# Autodesk Inventor assembly: CrossBot
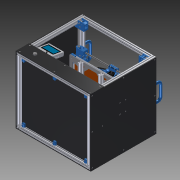
[picture p0: Inventor's stored thumbnail of the model, 180x180]
Saved by Autodesk Inventor 2015 SP1 (Build 190203100, 203)
## iProperties
Created: 2014-08-14
Part Number: CrossBot
Document SubType Name: Assembly
Designer: t_clevj
Mass: 16815.8 g
Surface Area: 53062.5 cm^2
Volume: 10946.1 cm^3
Density: 1.53623 g/cm^3
Author: t_clevj
## Documents named in this file (25)
- C:\Users\Jack\ownCloud\Projects\CrossBot\InventorModel\CrossBot.iam
- C:\Users\Jack\ownCloud\Projects\CrossBot\InventorModel\Frame\Frame.iam
- C:\Users\Jack\ownCloud\Projects\CrossBot\InventorModel\Hardware\Shaft\Shaft8\YShaft.ipt
- C:\Users\Jack\ownCloud\Projects\CrossBot\InventorModel\YAxis\YAxisMotorLeft.iam
- C:\Users\Jack\ownCloud\Projects\CrossBot\InventorModel\YAxis\YAxisIdlerLeft.iam
- C:\Users\Jack\ownCloud\Projects\CrossBot\InventorModel\YAxis\YAxisMotorRight.iam
- C:\Users\Jack\ownCloud\Projects\CrossBot\InventorModel\XAxis\XEndLeft.iam
- C:\Users\Jack\ownCloud\Projects\CrossBot\InventorModel\YAxis\YAxisIdlerRight.iam
- C:\Users\Jack\ownCloud\Projects\CrossBot\InventorModel\XAxis\XEndRight.iam
- C:\Users\Jack\ownCloud\Projects\CrossBot\InventorModel\Hardware\Shaft\Shaft8\XShaft.ipt
- C:\Users\Jack\ownCloud\Projects\CrossBot\InventorModel\Hardware\Shaft\Shaft10\ZAxisShaft.ipt
- C:\Users\Jack\ownCloud\Projects\CrossBot\InventorModel\Enclosure\SpoolFilament.ipt
- C:\Users\Jack\ownCloud\Projects\CrossBot\InventorModel\XAxis\XCarriage.iam
- C:\Users\Jack\ownCloud\Projects\CrossBot\InventorModel\Electronics\PSUUltibots.ipt
- C:\Users\Jack\ownCloud\Projects\CrossBot\InventorModel\Extruder\SanladererBowdenExtruder\SanladererBowdenExtruder.iam
- C:\Users\Jack\ownCloud\Projects\CrossBot\InventorModel\Extruder\SanladererBowdenExtruder\SanladererBowdenExtruderMirrored.iam
- C:\Users\Jack\ownCloud\Projects\CrossBot\InventorModel\ZAxis\ZAxisBed.iam
- C:\Users\Jack\ownCloud\Projects\CrossBot\InventorModel\ZAxis\ZAxisRodClamp.iam
- C:\Users\Jack\ownCloud\Projects\CrossBot\InventorModel\ZAxis\ZDrive.iam
- C:\Users\Jack\ownCloud\Projects\CrossBot\InventorModel\Electronics\KeySwitch\KeySwitch.iam
- C:\Users\Jack\ownCloud\Projects\CrossBot\InventorModel\ZAxis\ZEndstop.iam
- C:\Users\Jack\ownCloud\Projects\CrossBot\InventorModel\Electronics\Ports\PowerSocket.ipt
- C:\Users\Jack\ownCloud\Projects\CrossBot\InventorModel\Hardware\Nuts\ExtrusionNuts\ExtrusionNutHNKK5_4.ipt
- C:\Users\Jack\ownCloud\Projects\CrossBot\InventorModel\Electronics\Boards\RumbaBoard.ipt
- C:\Users\Jack\ownCloud\Projects\CrossBot\InventorModel\Enclosure\LCDCase\LCD+Case.iam
## Components (60 placed, 24 different names)
1. Frame:1 [sub-assembly] — Mate:6, Mate:23, Mate:24, Mate:25, Mate:27, Mate:28, Mate:29, Mate:30, Mate:31, Mate:32, Mate:69, Mate:70, Angle:13, Mate:260, Flush:89, Mate:261, Flush:90, Flush:92, Flush:93, Flush:94, Flush:95, Mate:352, Mate:353, Mate:354, Mate:355, Flush:98, Mate:381, Mate:382, Mate:383, Mate:400, Mate:401, Mate:402, Angle:46, Mate:417, Mate:418, Mate:419, Mate:426, Mate:427, Mate:428, Angle:47, Mate:465, Angle:50, Angle:51, Angle:52, Angle:53, Angle:54, Angle:55, Mate:466, Mate:467, Mate:468, Mate:469, Mate:470, Angle:56, Angle:58, Angle:59, Angle:60, Angle:61, Angle:62, Angle:63, Angle:64, Angle:65, Angle:66, Mate:471, Mate:472, Mate:473, Mate:474, Mate:475, Mate:476, Mate:477, Mate:478, Mate:479, Mate:480, Angle:67, Angle:68, Angle:69, Angle:70, Mate:481, Mate:482, Mate:483, Mate:484, Angle:71, Angle:72, Angle:73, Angle:74, Mate:485, Mate:486, Mate:487, Mate:488, Angle:75, Angle:76, Angle:77, Angle:78, Mate:489, Mate:490, Mate:491, Mate:492, Mate:497, Mate:498, Mate:499, Angle:79
2. RumbaBoard:1 — Mate:498
3. LCD+Case:1 [sub-assembly] — Mate:499, Angle:79
4. ZEndstop:1 [sub-assembly] — Mate:415, Angle:46, Mate:416
5. ZDrive:1 [sub-assembly] — Mate:381, Mate:382, Mate:383, Mate:384, Mate:431, Mate:459, Mate:460, Mate:461, Mate:462
6. ZAxisRodClamp:4 [sub-assembly] — Mate:350, Flush:95, Mate:355, Mate:384, Mate:455, Mate:456
7. ZAxisRodClamp:3 [sub-assembly] — Mate:349, Flush:94, Mate:352, Flush:97, Mate:416, Mate:463, Mate:464
8. ZAxisRodClamp:2 [sub-assembly] — Mate:348, Flush:92, Mate:354, Mate:457, Mate:458
9. ZAxisRodClamp:1 [sub-assembly] — Mate:347, Flush:93, Mate:353, Flush:96, Mate:449, Mate:450
10. ZAxisBed:1 [sub-assembly] — Mate:431, Angle:47
11. ZAxisShaft:1 — Mate:349, Mate:350, Mate:351, Flush:97, Mate:415
12. ZAxisShaft:2 — Mate:347, Mate:348, Mate:351, Flush:96
13. YShaft:2 — Mate:26, Mate:130, Mate:514
14. YShaft:3 — Mate:37, Mate:190
15. YAxisMotorLeft:1 [sub-assembly] — Mate:23, Mate:24, Mate:25, Mate:26, Mate:439, Mate:440, Mate:441, Mate:442
16. YAxisMotorRight:1 [sub-assembly] — Mate:30, Mate:31, Mate:32, Mate:37, Mate:435, Mate:436, Mate:437, Mate:438
17. YAxisIdlerLeft:1 [sub-assembly] — Mate:27, Mate:28, Mate:29, Mate:130, Mate:443, Mate:444, Mate:445
18. YAxisIdlerRight:1 [sub-assembly] — Mate:426, Mate:427, Mate:428, Mate:446, Mate:447, Mate:448
19. XShaft:1 — Mate:189, Flush:54, Mate:513, Mate:515
20. XShaft:2 — Mate:188, Flush:55, Mate:191, Mate:516
21. XCarriage:1 [sub-assembly] — Mate:515, Mate:516
22. XEndLeft:1 [sub-assembly] — Mate:188, Mate:189, Flush:54, Flush:55, Mate:514
23. XEndRight:1 [sub-assembly] — Mate:190, Mate:191, Angle:13, Mate:513
24. KeySwitch:1 [sub-assembly] — Mate:400, Mate:401, Mate:402
25. PowerSocket:1 — Mate:417, Mate:418, Mate:419
26. PSUUltibots:1 — Mate:497
27. SpoolFilament:3 — Mate:504
28. SpoolFilament:4 — Mate:504
29. SanladererBowdenExtruderMirrored:1 [sub-assembly] — Mate:261, Flush:90, Flush:91, Mate:493, Mate:494
30. SanladererBowdenExtruder:1 [sub-assembly] — Mate:260, Flush:89, Flush:91, Flush:98, Mate:495, Mate:496
31. ExtrusionNutHNKK5_4:22 — Mate:455, Angle:51, Mate:469
32. ExtrusionNutHNKK5_4:30 — Mate:464, Angle:74, Mate:485
33. ExtrusionNutHNKK5_4:29 — Mate:463, Angle:71, Mate:486
34. ExtrusionNutHNKK5_4:16 — Mate:450, Angle:73, Mate:487
35. ExtrusionNutHNKK5_4:15 — Mate:449, Angle:72, Mate:488
36. ExtrusionNutHNKK5_4:23 — Mate:457, Angle:53, Mate:466
37. ExtrusionNutHNKK5_4:24 — Mate:458, Angle:54, Mate:470
38. ExtrusionNutHNKK5_4:21 — Mate:456, Mate:465, Angle:50
39. ExtrusionNutHNKK5_4:28 — Mate:462, Angle:55, Mate:468
40. ExtrusionNutHNKK5_4:27 — Mate:461, Angle:52, Mate:467
41. ExtrusionNutHNKK5_4:26 — Mate:459
42. ExtrusionNutHNKK5_4:25 — Mate:460
43. ExtrusionNutHNKK5_4:4 — Mate:438, Angle:76, Mate:492
44. ExtrusionNutHNKK5_4:1 — Mate:437, Angle:61, Mate:476
45. ExtrusionNutHNKK5_4:2 — Mate:436, Angle:63, Mate:474
46. ExtrusionNutHNKK5_4:3 — Mate:435, Angle:62, Mate:475
47. ExtrusionNutHNKK5_4:5 — Mate:442, Angle:75, Mate:491
48. ExtrusionNutHNKK5_4:6 — Mate:441, Angle:66, Mate:471
49. ExtrusionNutHNKK5_4:8 — Mate:439, Angle:64, Mate:473
50. ExtrusionNutHNKK5_4:7 — Mate:440, Angle:65, Mate:472
51. ExtrusionNutHNKK5_4:14 — Mate:448, Angle:78, Mate:489
52. ExtrusionNutHNKK5_4:12 — Mate:446, Angle:60, Mate:477
53. ExtrusionNutHNKK5_4:13 — Mate:447, Angle:56, Mate:478
54. ExtrusionNutHNKK5_4:10 — Mate:443, Angle:58, Mate:479
55. ExtrusionNutHNKK5_4:11 — Mate:445, Angle:59, Mate:480
56. ExtrusionNutHNKK5_4:9 — Mate:444, Angle:77, Mate:490
57. ExtrusionNutHNKK5_4:18 — Angle:67, Mate:483, Mate:493
58. ExtrusionNutHNKK5_4:17 — Angle:68, Mate:484, Mate:494
59. ExtrusionNutHNKK5_4:20 — Angle:69, Mate:481, Mate:496
60. ExtrusionNutHNKK5_4:19 — Angle:70, Mate:482, Mate:495
## Relationships (156: Mate 112, Angle 32, Flush 12)
- Mate:6: Frame:1
- Mate:23: Frame:1 ↔ YAxisMotorLeft:1
- Mate:24: Frame:1 ↔ YAxisMotorLeft:1
- Mate:25: Frame:1 ↔ YAxisMotorLeft:1
- Mate:26: YShaft:2 ↔ YAxisMotorLeft:1
- Mate:27: Frame:1 ↔ YAxisIdlerLeft:1
- Mate:28: Frame:1 ↔ YAxisIdlerLeft:1
- Mate:29: Frame:1 ↔ YAxisIdlerLeft:1
- Mate:30: Frame:1 ↔ YAxisMotorRight:1
- Mate:31: Frame:1 ↔ YAxisMotorRight:1
- Mate:32: Frame:1 ↔ YAxisMotorRight:1
- Mate:37: YShaft:3 ↔ YAxisMotorRight:1
- Mate:69: Frame:1
- Mate:70: Frame:1
- Mate:130: YShaft:2 ↔ YAxisIdlerLeft:1
- Mate:188: XShaft:2 ↔ XEndLeft:1
- Mate:189: XShaft:1 ↔ XEndLeft:1
- Flush:54: XShaft:1 ↔ XEndLeft:1
- Flush:55: XShaft:2 ↔ XEndLeft:1
- Mate:190: YShaft:3 ↔ XEndRight:1
- Mate:191: XShaft:2 ↔ XEndRight:1
- Angle:13 (0 deg): Frame:1 ↔ XEndRight:1
- Mate:260: Frame:1 ↔ SanladererBowdenExtruder:1
- Flush:89 (2 mm): Frame:1 ↔ SanladererBowdenExtruder:1
- Mate:261: Frame:1 ↔ SanladererBowdenExtruderMirrored:1
- Flush:90 (2 mm): Frame:1 ↔ SanladererBowdenExtruderMirrored:1
- Flush:91: SanladererBowdenExtruderMirrored:1 ↔ SanladererBowdenExtruder:1
- Mate:347: ZAxisRodClamp:1 ↔ ZAxisShaft:2
- Mate:348: ZAxisRodClamp:2 ↔ ZAxisShaft:2
- Flush:92: Frame:1 ↔ ZAxisRodClamp:2
- Flush:93: Frame:1 ↔ ZAxisRodClamp:1
- Mate:349: ZAxisRodClamp:3 ↔ ZAxisShaft:1
- Flush:94: Frame:1 ↔ ZAxisRodClamp:3
- Mate:350: ZAxisRodClamp:4 ↔ ZAxisShaft:1
- Flush:95: Frame:1 ↔ ZAxisRodClamp:4
- Mate:351 (130 mm): ZAxisShaft:1 ↔ ZAxisShaft:2
- Mate:352: Frame:1 ↔ ZAxisRodClamp:3
- Mate:353: Frame:1 ↔ ZAxisRodClamp:1
- Mate:354: Frame:1 ↔ ZAxisRodClamp:2
- Mate:355: Frame:1 ↔ ZAxisRodClamp:4
- Flush:96: ZAxisRodClamp:1 ↔ ZAxisShaft:2
- Flush:97: ZAxisRodClamp:3 ↔ ZAxisShaft:1
- Flush:98 (82 mm): Frame:1 ↔ SanladererBowdenExtruder:1
- Mate:381: Frame:1 ↔ ZDrive:1
- Mate:382: Frame:1 ↔ ZDrive:1
- Mate:383 (187.5 mm): Frame:1 ↔ ZDrive:1
- Mate:384 (24.5 mm): ZDrive:1 ↔ ZAxisRodClamp:4
- Mate:400: Frame:1 ↔ KeySwitch:1
- Mate:401: Frame:1 ↔ KeySwitch:1
- Mate:402: Frame:1 ↔ KeySwitch:1
- Mate:415: ZEndstop:1 ↔ ZAxisShaft:1
- Angle:46 (0 deg): Frame:1 ↔ ZEndstop:1
- Mate:416 (6.5 mm): ZEndstop:1 ↔ ZAxisRodClamp:3
- Mate:417: Frame:1 ↔ PowerSocket:1
- Mate:418: Frame:1 ↔ PowerSocket:1
- Mate:419: Frame:1 ↔ PowerSocket:1
- Mate:426: Frame:1 ↔ YAxisIdlerRight:1
- Mate:427: Frame:1 ↔ YAxisIdlerRight:1
- Mate:428: Frame:1 ↔ YAxisIdlerRight:1
- Mate:431: ZDrive:1 ↔ ZAxisBed:1
- Angle:47 (0 deg): Frame:1 ↔ ZAxisBed:1
- Mate:435: YAxisMotorRight:1 ↔ ExtrusionNutHNKK5_4:3
- Mate:436: YAxisMotorRight:1 ↔ ExtrusionNutHNKK5_4:2
- Mate:437: YAxisMotorRight:1 ↔ ExtrusionNutHNKK5_4:1
- Mate:438: YAxisMotorRight:1 ↔ ExtrusionNutHNKK5_4:4
- Mate:439: YAxisMotorLeft:1 ↔ ExtrusionNutHNKK5_4:8
- Mate:440: YAxisMotorLeft:1 ↔ ExtrusionNutHNKK5_4:7
- Mate:441: YAxisMotorLeft:1 ↔ ExtrusionNutHNKK5_4:6
- Mate:442: YAxisMotorLeft:1 ↔ ExtrusionNutHNKK5_4:5
- Mate:443: YAxisIdlerLeft:1 ↔ ExtrusionNutHNKK5_4:10
- Mate:444: YAxisIdlerLeft:1 ↔ ExtrusionNutHNKK5_4:9
- Mate:445: YAxisIdlerLeft:1 ↔ ExtrusionNutHNKK5_4:11
- Mate:446: YAxisIdlerRight:1 ↔ ExtrusionNutHNKK5_4:12
- Mate:447: YAxisIdlerRight:1 ↔ ExtrusionNutHNKK5_4:13
- Mate:448: YAxisIdlerRight:1 ↔ ExtrusionNutHNKK5_4:14
- Mate:449: ZAxisRodClamp:1 ↔ ExtrusionNutHNKK5_4:15
- Mate:450: ZAxisRodClamp:1 ↔ ExtrusionNutHNKK5_4:16
- Mate:455: ZAxisRodClamp:4 ↔ ExtrusionNutHNKK5_4:22
- Mate:456: ZAxisRodClamp:4 ↔ ExtrusionNutHNKK5_4:21
- Mate:457: ZAxisRodClamp:2 ↔ ExtrusionNutHNKK5_4:23
- Mate:458: ZAxisRodClamp:2 ↔ ExtrusionNutHNKK5_4:24
- Mate:459: ZDrive:1 ↔ ExtrusionNutHNKK5_4:26
- Mate:460: ZDrive:1 ↔ ExtrusionNutHNKK5_4:25
- Mate:461: ZDrive:1 ↔ ExtrusionNutHNKK5_4:27
- Mate:462: ZDrive:1 ↔ ExtrusionNutHNKK5_4:28
- Mate:463: ZAxisRodClamp:3 ↔ ExtrusionNutHNKK5_4:29
- Mate:464: ZAxisRodClamp:3 ↔ ExtrusionNutHNKK5_4:30
- Mate:465: Frame:1 ↔ ExtrusionNutHNKK5_4:21
- Angle:50 (0 deg): Frame:1 ↔ ExtrusionNutHNKK5_4:21
- Angle:51 (0 deg): Frame:1 ↔ ExtrusionNutHNKK5_4:22
- Angle:52 (0 deg): Frame:1 ↔ ExtrusionNutHNKK5_4:27
- Angle:53 (0 deg): Frame:1 ↔ ExtrusionNutHNKK5_4:23
- Angle:54 (0 deg): Frame:1 ↔ ExtrusionNutHNKK5_4:24
- Angle:55 (0 deg): Frame:1 ↔ ExtrusionNutHNKK5_4:28
- Mate:466: Frame:1 ↔ ExtrusionNutHNKK5_4:23
- Mate:467: Frame:1 ↔ ExtrusionNutHNKK5_4:27
- Mate:468: Frame:1 ↔ ExtrusionNutHNKK5_4:28
- Mate:469: Frame:1 ↔ ExtrusionNutHNKK5_4:22
- Mate:470: Frame:1 ↔ ExtrusionNutHNKK5_4:24
- Angle:56 (0 deg): Frame:1 ↔ ExtrusionNutHNKK5_4:13
- Angle:58 (0 deg): Frame:1 ↔ ExtrusionNutHNKK5_4:10
- Angle:59 (0 deg): Frame:1 ↔ ExtrusionNutHNKK5_4:11
- Angle:60 (0 deg): Frame:1 ↔ ExtrusionNutHNKK5_4:12
- Angle:61 (0 deg): Frame:1 ↔ ExtrusionNutHNKK5_4:1
- Angle:62 (0 deg): Frame:1 ↔ ExtrusionNutHNKK5_4:3
- Angle:63 (0 deg): Frame:1 ↔ ExtrusionNutHNKK5_4:2
- Angle:64 (0 deg): Frame:1 ↔ ExtrusionNutHNKK5_4:8
- Angle:65 (0 deg): Frame:1 ↔ ExtrusionNutHNKK5_4:7
- Angle:66 (0 deg): Frame:1 ↔ ExtrusionNutHNKK5_4:6
- Mate:471: Frame:1 ↔ ExtrusionNutHNKK5_4:6
- Mate:472: Frame:1 ↔ ExtrusionNutHNKK5_4:7
- Mate:473: Frame:1 ↔ ExtrusionNutHNKK5_4:8
- Mate:474: Frame:1 ↔ ExtrusionNutHNKK5_4:2
- Mate:475: Frame:1 ↔ ExtrusionNutHNKK5_4:3
- Mate:476: Frame:1 ↔ ExtrusionNutHNKK5_4:1
- Mate:477: Frame:1 ↔ ExtrusionNutHNKK5_4:12
- Mate:478: Frame:1 ↔ ExtrusionNutHNKK5_4:13
- Mate:479: Frame:1 ↔ ExtrusionNutHNKK5_4:10
- Mate:480: Frame:1 ↔ ExtrusionNutHNKK5_4:11
- Angle:67 (0 deg): Frame:1 ↔ ExtrusionNutHNKK5_4:18
- Angle:68 (0 deg): Frame:1 ↔ ExtrusionNutHNKK5_4:17
- Angle:69 (0 deg): Frame:1 ↔ ExtrusionNutHNKK5_4:20
- Angle:70 (0 deg): Frame:1 ↔ ExtrusionNutHNKK5_4:19
- Mate:481: Frame:1 ↔ ExtrusionNutHNKK5_4:20
- Mate:482: Frame:1 ↔ ExtrusionNutHNKK5_4:19
- Mate:483: Frame:1 ↔ ExtrusionNutHNKK5_4:18
- Mate:484: Frame:1 ↔ ExtrusionNutHNKK5_4:17
- Angle:71 (0 deg): Frame:1 ↔ ExtrusionNutHNKK5_4:29
- Angle:72 (0 deg): Frame:1 ↔ ExtrusionNutHNKK5_4:15
- Angle:73 (0 deg): Frame:1 ↔ ExtrusionNutHNKK5_4:16
- Angle:74 (0 deg): Frame:1 ↔ ExtrusionNutHNKK5_4:30
- Mate:485: Frame:1 ↔ ExtrusionNutHNKK5_4:30
- Mate:486: Frame:1 ↔ ExtrusionNutHNKK5_4:29
- Mate:487: Frame:1 ↔ ExtrusionNutHNKK5_4:16
- Mate:488: Frame:1 ↔ ExtrusionNutHNKK5_4:15
- Angle:75 (0 deg): Frame:1 ↔ ExtrusionNutHNKK5_4:5
- Angle:76 (0 deg): Frame:1 ↔ ExtrusionNutHNKK5_4:4
- Angle:77 (0 deg): Frame:1 ↔ ExtrusionNutHNKK5_4:9
- Angle:78 (0 deg): Frame:1 ↔ ExtrusionNutHNKK5_4:14
- Mate:489: Frame:1 ↔ ExtrusionNutHNKK5_4:14
- Mate:490: Frame:1 ↔ ExtrusionNutHNKK5_4:9
- Mate:491: Frame:1 ↔ ExtrusionNutHNKK5_4:5
- Mate:492: Frame:1 ↔ ExtrusionNutHNKK5_4:4
- Mate:493: SanladererBowdenExtruderMirrored:1 ↔ ExtrusionNutHNKK5_4:18
- Mate:494: SanladererBowdenExtruderMirrored:1 ↔ ExtrusionNutHNKK5_4:17
- Mate:495: SanladererBowdenExtruder:1 ↔ ExtrusionNutHNKK5_4:19
- Mate:496: SanladererBowdenExtruder:1 ↔ ExtrusionNutHNKK5_4:20
- Mate:497: Frame:1 ↔ PSUUltibots:1
- Mate:498: Frame:1 ↔ RumbaBoard:1
- Mate:499: Frame:1 ↔ LCD+Case:1
- Angle:79 (180 deg): Frame:1 ↔ LCD+Case:1
- Mate:504: SpoolFilament:3 ↔ SpoolFilament:4
- Mate:513: XShaft:1 ↔ XEndRight:1
- Mate:514: YShaft:2 ↔ XEndLeft:1
- Mate:515: XShaft:1 ↔ XCarriage:1
- Mate:516: XShaft:2 ↔ XCarriage:1
